# Autodesk Inventor assembly: Frame
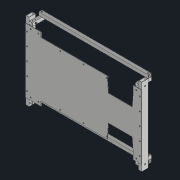
[picture p0: Inventor's stored thumbnail of the model, 180x180]
Saved by Autodesk Inventor 2022 (Build 260153000, 153)
## iProperties
Created: 2022-09-10
Part Number: Frame
Document SubType Name: Assembly
Designer: robpl
Author: robpl
## Documents named in this file (9)
- C:\Users\robpl\OneDrive\Documents\Inventor\2022 FRC Season\Best Coast Drive\Frame.iam
- C:\Users\robpl\OneDrive\Documents\Inventor\2022 FRC Season\Best Coast Drive\Bellypan.ipt
- C:\Users\robpl\OneDrive\Documents\Inventor\2022 FRC Season\Best Coast Drive\Front Bar.ipt
- C:\Users\robpl\OneDrive\Documents\Inventor\2022 FRC Season\Best Coast Drive\M5 x 12.7 Rivet.ipt
- C:\Users\robpl\OneDrive\Documents\Inventor\2022 FRC Season\Best Coast Drive\Back Bar.ipt
- C:\Users\robpl\OneDrive\Documents\Inventor\2022 FRC Season\Best Coast Drive\Side Bar Mount.ipt
- C:\Users\robpl\OneDrive\Documents\Inventor\2022 FRC Season\Best Coast Drive\Side Bar.ipt
- C:\Users\robpl\OneDrive\Documents\Inventor\Content Center Files\R2022\en-US\ISO 4762(2)\ISO 4762 - M6 x 40ISO.ipt
- C:\Users\robpl\OneDrive\Documents\Inventor\Content Center Files\R2022\en-US\ISO 7041\ISO 7041 - M6 - ISO.ipt
## Components (47 placed, 8 different names)
1. Bellypan:1 — Mate:1, Mate:2, Mate:3, Mate:4, Mate:5, Mate:6, Mate:7, Mate:8, Mate:9, Mate:10, Mate:11, Mate:12, Mate:13, Mate:14, Mate:17, Mate:18, Mate:19, Mate:20
2. Front Bar:1 — Mate:1, Mate:2, Mate:5, Mate:22, Mate:23, Mate:25, Mate:26, Mate:49, Mate:50, Mate:51, Mate:52, Mate:53, Mate:55
3. Back Bar:1 — Mate:12, Mate:13, Mate:14, Mate:15, Mate:16, Mate:21, Mate:24, Mate:33, Mate:34, Mate:35, Mate:36, Mate:37, Mate:39
4. Side Bar Mount:1 — Mate:20, Mate:21, Mate:24, Mate:29, Mate:38, Mate:40, Mate:46, Mate:48
5. Side Bar Mount:2 — Mate:15, Mate:16, Mate:17, Mate:30, Mate:31
6. Side Bar Mount:3 — Mate:18, Mate:23, Mate:25, Mate:27, Mate:28, Mate:54, Mate:56
7. Side Bar Mount:4 — Mate:19, Mate:22, Mate:26, Mate:32, Mate:62, Mate:64
8. Side Bar:1 — Mate:27, Mate:28, Mate:29, Mate:41, Mate:42, Mate:43, Mate:44, Mate:45, Mate:47
9. Side Bar:2 — Mate:30, Mate:31, Mate:32, Mate:57, Mate:58, Mate:59, Mate:60, Mate:61, Mate:63
10. ISO 4762 M6 x 40:1 — Mate:33, Mate:34
11. ISO 7041 M6:1 — Mate:37, Mate:38
12. ISO 4762 M6 x 40:2 — Mate:35, Mate:36
13. ISO 7041 M6:2 — Mate:39, Mate:40
14. ISO 4762 M6 x 40:3 — Mate:41, Mate:42
15. ISO 7041 M6:3 — Mate:45, Mate:46
16. ISO 4762 M6 x 40:4 — Mate:43, Mate:44
17. ISO 7041 M6:4 — Mate:47, Mate:48
18. ISO 4762 M6 x 40:5 — Mate:49, Mate:50
19. ISO 7041 M6:5 — Mate:53, Mate:54
20. ISO 4762 M6 x 40:6 — Mate:51, Mate:52
21. ISO 7041 M6:6 — Mate:55, Mate:56
22. ISO 4762 M6 x 40:7 — Mate:57, Mate:58
23. ISO 7041 M6:7 — Mate:61, Mate:62
24. ISO 4762 M6 x 40:8 — Mate:59, Mate:60
25. ISO 7041 M6:8 — Mate:63, Mate:64
26. M5 x 12.7 Rivet:1 — Mate:3, Mate:4
27. M5 x 12.7 Rivet:2
28. M5 x 12.7 Rivet:3
29. M5 x 12.7 Rivet:4
30. M5 x 12.7 Rivet:5
31. M5 x 12.7 Rivet:6
32. M5 x 12.7 Rivet:7
33. M5 x 12.7 Rivet:8
34. M5 x 12.7 Rivet:9
35. M5 x 12.7 Rivet:10
36. M5 x 12.7 Rivet:11 — Mate:6, Mate:7
37. M5 x 12.7 Rivet:12
38. M5 x 12.7 Rivet:13
39. M5 x 12.7 Rivet:14
40. M5 x 12.7 Rivet:15 — Mate:8, Mate:9
41. M5 x 12.7 Rivet:17
42. M5 x 12.7 Rivet:18
43. M5 x 12.7 Rivet:19
44. M5 x 12.7 Rivet:20
45. M5 x 12.7 Rivet:21
46. M5 x 12.7 Rivet:16 — Mate:10, Mate:11
47. M5 x 12.7 Rivet:22
## Component patterns: (10 elements, first: M5 x 12.7 Rivet:1), (4 elements, first: M5 x 12.7 Rivet:11), (6 elements, first: M5 x 12.7 Rivet:15), (2 elements, first: M5 x 12.7 Rivet:16)
## Relationships (64: Mate 64)
- Mate:1: Bellypan:1 ↔ Front Bar:1
- Mate:2: Bellypan:1 ↔ Front Bar:1
- Mate:3: Bellypan:1 ↔ M5 x 12.7 Rivet:1
- Mate:4: Bellypan:1 ↔ M5 x 12.7 Rivet:1
- Mate:5: Bellypan:1 ↔ Front Bar:1
- Mate:6: Bellypan:1 ↔ M5 x 12.7 Rivet:11
- Mate:7: Bellypan:1 ↔ M5 x 12.7 Rivet:11
- Mate:8: Bellypan:1 ↔ M5 x 12.7 Rivet:15
- Mate:9: Bellypan:1 ↔ M5 x 12.7 Rivet:15
- Mate:10: Bellypan:1 ↔ M5 x 12.7 Rivet:16
- Mate:11: Bellypan:1 ↔ M5 x 12.7 Rivet:16
- Mate:12: Bellypan:1 ↔ Back Bar:1
- Mate:13: Bellypan:1 ↔ Back Bar:1
- Mate:14: Bellypan:1 ↔ Back Bar:1
- Mate:15: Back Bar:1 ↔ Side Bar Mount:2
- Mate:16: Back Bar:1 ↔ Side Bar Mount:2
- Mate:17: Bellypan:1 ↔ Side Bar Mount:2
- Mate:18: Bellypan:1 ↔ Side Bar Mount:3
- Mate:19: Bellypan:1 ↔ Side Bar Mount:4
- Mate:20: Bellypan:1 ↔ Side Bar Mount:1
- Mate:21: Back Bar:1 ↔ Side Bar Mount:1
- Mate:22: Front Bar:1 ↔ Side Bar Mount:4
- Mate:23: Front Bar:1 ↔ Side Bar Mount:3
- Mate:24: Back Bar:1 ↔ Side Bar Mount:1
- Mate:25: Front Bar:1 ↔ Side Bar Mount:3
- Mate:26: Front Bar:1 ↔ Side Bar Mount:4
- Mate:27: Side Bar Mount:3 ↔ Side Bar:1
- Mate:28: Side Bar Mount:3 ↔ Side Bar:1
- Mate:29: Side Bar Mount:1 ↔ Side Bar:1
- Mate:30: Side Bar Mount:2 ↔ Side Bar:2
- Mate:31: Side Bar Mount:2 ↔ Side Bar:2
- Mate:32: Side Bar Mount:4 ↔ Side Bar:2
- Mate:33: Back Bar:1 ↔ ISO 4762 M6 x 40:1
- Mate:34: Back Bar:1 ↔ ISO 4762 M6 x 40:1
- Mate:35: Back Bar:1 ↔ ISO 4762 M6 x 40:2
- Mate:36: Back Bar:1 ↔ ISO 4762 M6 x 40:2
- Mate:37: Back Bar:1 ↔ ISO 7041 M6:1
- Mate:38: Side Bar Mount:1 ↔ ISO 7041 M6:1
- Mate:39: Back Bar:1 ↔ ISO 7041 M6:2
- Mate:40: Side Bar Mount:1 ↔ ISO 7041 M6:2
- Mate:41: Side Bar:1 ↔ ISO 4762 M6 x 40:3
- Mate:42: Side Bar:1 ↔ ISO 4762 M6 x 40:3
- Mate:43: Side Bar:1 ↔ ISO 4762 M6 x 40:4
- Mate:44: Side Bar:1 ↔ ISO 4762 M6 x 40:4
- Mate:45: Side Bar:1 ↔ ISO 7041 M6:3
- Mate:46: Side Bar Mount:1 ↔ ISO 7041 M6:3
- Mate:47: Side Bar:1 ↔ ISO 7041 M6:4
- Mate:48: Side Bar Mount:1 ↔ ISO 7041 M6:4
- Mate:49: Front Bar:1 ↔ ISO 4762 M6 x 40:5
- Mate:50: Front Bar:1 ↔ ISO 4762 M6 x 40:5
- Mate:51: Front Bar:1 ↔ ISO 4762 M6 x 40:6
- Mate:52: Front Bar:1 ↔ ISO 4762 M6 x 40:6
- Mate:53: Front Bar:1 ↔ ISO 7041 M6:5
- Mate:54: Side Bar Mount:3 ↔ ISO 7041 M6:5
- Mate:55: Front Bar:1 ↔ ISO 7041 M6:6
- Mate:56: Side Bar Mount:3 ↔ ISO 7041 M6:6
- Mate:57: Side Bar:2 ↔ ISO 4762 M6 x 40:7
- Mate:58: Side Bar:2 ↔ ISO 4762 M6 x 40:7
- Mate:59: Side Bar:2 ↔ ISO 4762 M6 x 40:8
- Mate:60: Side Bar:2 ↔ ISO 4762 M6 x 40:8
- Mate:61: Side Bar:2 ↔ ISO 7041 M6:7
- Mate:62: Side Bar Mount:4 ↔ ISO 7041 M6:7
- Mate:63: Side Bar:2 ↔ ISO 7041 M6:8
- Mate:64: Side Bar Mount:4 ↔ ISO 7041 M6:8
